# Autodesk Inventor assembly: 00_XY_stage-CHUO_SEIKI_LD-647-R1
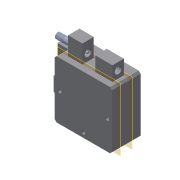
[picture p0: Inventor's stored thumbnail of the model, 180x180]
Saved by Autodesk Inventor 2019 (Build 230136000, 136)
## iProperties
Created: 2019-05-02
Part Number: 00_XY_stage-CHUO_SEIKI_LD-647-R1
Document SubType Name: Assembly
Designer: diederichbenedict
Author: diederichbenedict
## Documents named in this file (5)
- C:\Users\diederichbenedict\Dropbox\Dokumente\Promotion\PROJECTS\STORMoChip\INVENTOR\Nanoscopy-on-a-cheap\00_XY_stage-Chinese_60x60-R1.iam
- C:\Users\diederichbenedict\Dropbox\Dokumente\Promotion\PROJECTS\STORMoChip\INVENTOR\Nanoscopy-on-a-cheap\00_XY_stage-CHUO_SEIKI_LD-647-R1-Micrometer.ipt
- C:\Users\diederichbenedict\Dropbox\Dokumente\Promotion\PROJECTS\STORMoChip\INVENTOR\Nanoscopy-on-a-cheap\00_XY_stage-Chinese_60x60-R1-Top.ipt
- C:\Users\diederichbenedict\Dropbox\Dokumente\Promotion\PROJECTS\STORMoChip\INVENTOR\Nanoscopy-on-a-cheap\00_XY_stage-Chinese_60x60-R1-Middle.ipt
- C:\Users\diederichbenedict\Dropbox\Dokumente\Promotion\PROJECTS\STORMoChip\INVENTOR\Nanoscopy-on-a-cheap\00_XY_stage-Chinese_60x60-R1-Bottom.ipt
## Components (5 placed, 4 different names)
1. 00_XY_stage-Chinese_60x60-R1-Top:1 — Flush:1, Flush:2, Insert:2
2. 00_XY_stage-Chinese_60x60-R1-Middle:1 — Flush:1, Flush:2, Flush:3, Flush:4, Insert:3
3. 00_XY_stage-Chinese_60x60-R1-Bottom:1 — Flush:3, Flush:4
4. 00_XY_stage-CHUO_SEIKI_LD-647-R1-Micrometer:3 — Insert:2
5. 00_XY_stage-CHUO_SEIKI_LD-647-R1-Micrometer:4 — Insert:3
## Relationships (6: Flush 4, Insert 2)
- Flush:1: 00_XY_stage-Chinese_60x60-R1-Top:1 ↔ 00_XY_stage-Chinese_60x60-R1-Middle:1
- Flush:2: 00_XY_stage-Chinese_60x60-R1-Top:1 ↔ 00_XY_stage-Chinese_60x60-R1-Middle:1
- Flush:3: 00_XY_stage-Chinese_60x60-R1-Middle:1 ↔ 00_XY_stage-Chinese_60x60-R1-Bottom:1
- Flush:4: 00_XY_stage-Chinese_60x60-R1-Middle:1 ↔ 00_XY_stage-Chinese_60x60-R1-Bottom:1
- Insert:2: 00_XY_stage-Chinese_60x60-R1-Top:1 ↔ 00_XY_stage-CHUO_SEIKI_LD-647-R1-Micrometer:3
- Insert:3: 00_XY_stage-Chinese_60x60-R1-Middle:1 ↔ 00_XY_stage-CHUO_SEIKI_LD-647-R1-Micrometer:4
